# Autodesk Inventor assembly: Optics Assembly
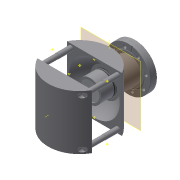
[picture p0: Inventor's stored thumbnail of the model, 180x180]
Saved by Autodesk Inventor 2015 (Build 190159000, 159)
## iProperties
Created: 2014-07-17
Part Number: Optics Assembly
Document SubType Name: Assembly
Designer: I Rabey
Author: I Rabey
## Documents named in this file (6)
- C:\CADFiles\EDM Machine\Detection Region\Re-entrant Flange and Mirrors\Optics Assembly.iam
- C:\CADFiles\EDM Machine\Detection Region\Re-entrant Flange and Mirrors\Mirrors\Ideas\Mirror Assembly.iam
- C:\CADFiles\EDM Machine\Detection Region\Re-entrant Flange and Mirrors\Re-entrant Flange.iam
- C:\CADFiles\EDM Machine\Detection Region\Re-entrant Flange and Mirrors\Mirrors\Custom Mirror Design.ipt
- C:\CADFiles\EDM Machine\Detection Region\Re-entrant Flange and Mirrors\Mirrors\Custom Mirror Design Part 2.ipt
- C:\CADFiles\EDM Machine\Detection Region\Re-entrant Flange and Mirrors\holdingRod.ipt
## Components (8 placed, 5 different names)
1. Mirror Assembly:1 [sub-assembly]
2. Re-entrant Flange:1 [sub-assembly] — Mate:20, Mate:21, Mate:25, Mate:30
3. Custom Mirror Design:1 — Mate:25, Mate:31, Mate:32
4. Custom Mirror Design Part 2:1 — Mate:21, Mate:27, Insert:1, Insert:2, Insert:3, Mate:29, Mate:30, Angle:1, Mate:32
5. holdingRod:1 — Insert:3
6. holdingRod:2 — Insert:1, Mate:31
7. holdingRod:3 — Insert:2
8. holdingRod:4 — Mate:29
## Relationships (14: Mate 10, Insert 3, Angle 1)
- Mate:11
- Mate:12
- Mate:20: Re-entrant Flange:1
- Mate:21: Re-entrant Flange:1 ↔ Custom Mirror Design Part 2:1
- Mate:25: Re-entrant Flange:1 ↔ Custom Mirror Design:1
- Mate:27 (75 mm): Custom Mirror Design Part 2:1
- Insert:1: Custom Mirror Design Part 2:1 ↔ holdingRod:2
- Insert:2: Custom Mirror Design Part 2:1 ↔ holdingRod:3
- Insert:3: Custom Mirror Design Part 2:1 ↔ holdingRod:1
- Mate:29: Custom Mirror Design Part 2:1 ↔ holdingRod:4
- Mate:30: Re-entrant Flange:1 ↔ Custom Mirror Design Part 2:1
- Mate:31: Custom Mirror Design:1 ↔ holdingRod:2
- Angle:1 (0 deg): Custom Mirror Design Part 2:1
- Mate:32 (75.75 mm): Custom Mirror Design:1 ↔ Custom Mirror Design Part 2:1
